# Autodesk Inventor assembly: Нога левая в сборе
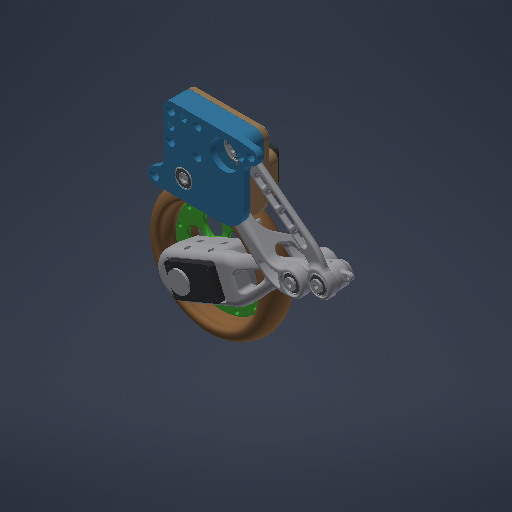
[picture p0: Inventor's stored thumbnail of the model, 512x512]
Saved by Autodesk Inventor 2025 (Build 290162010, 162A)
## iProperties
Created: 2024-06-21
Part Number: Нога левая в сборе
Document SubType Name: Assembly
Designer: Edward_Higgins
Author: Edward_Higgins
## Documents named in this file (14)
- D:\Users\Edward_Higgins\Desktop\ZAVOD\TWR2\Нога левая в сборе 2.iam
- D:\Users\Edward_Higgins\Desktop\ZAVOD\TWR2\Тяга передняя.ipt
- D:\Users\Edward_Higgins\Desktop\ZAVOD\TWR2\Стандартные детали\DYNAMIXEL XM430-W350.ipt
- D:\Users\Edward_Higgins\Desktop\ZAVOD\TWR2\Тяга задняя 2.ipt
- D:\Users\Edward_Higgins\Desktop\ZAVOD\TWR2\Голень в сборе.iam
- D:\Users\Edward_Higgins\Desktop\ZAVOD\TWR2\Стандартные детали\Подшипник.ipt
- D:\Users\Edward_Higgins\Desktop\ZAVOD\TWR2\Стопорная шайба.ipt
- D:\Users\Edward_Higgins\Desktop\ZAVOD\TWR2\Шайба.ipt
- D:\Users\Edward_Higgins\Desktop\ZAVOD\TWR2\Ось односторонняя.ipt
- D:\Users\Edward_Higgins\Desktop\ZAVOD\TWR2\Колесо 2 в сборе.iam
- D:\Users\Edward_Higgins\Desktop\ZAVOD\TWR2\Корпус ноги в сборе.iam
- D:\Users\Edward_Higgins\Desktop\ZAVOD\TWR2\Ось шарнира.ipt
- D:\Users\Edward_Higgins\Desktop\ZAVOD\TWR2\Ось двусторонняя.ipt
- D:\Users\Edward_Higgins\Desktop\ZAVOD\Робот Сколково\Нога левая в сборе\AIP\FEA\ew5x1yt6p.fres
## Components (19 placed, 12 different names)
1. Тяга передняя:1 — Совмещение:21, Совмещение:84, Совмещение:85, Совмещение:103, Совмещение:113, Совмещение:115, Совмещение:121, Совмещение:124, Совмещение:129, Совмещение:137
2. DYNAMIXEL XM430-W350:2 — Совмещение:21, Совмещение:84, Угол:1, Совмещение:104
3. Голень в сборе:1 [sub-assembly] — Совмещение:85, Совмещение:99, Совмещение:100, Совмещение:105, Совмещение:116, Совмещение:121, Совмещение:122
4. Подшипник:1 — Совмещение:110
5. Стопорная шайба:1
6. Шайба:1 — Совмещение:96, Совмещение:109
7. Ось односторонняя:1 — Совмещение:96, Совмещение:107, Совмещение:108
8. Колесо 2 в сборе:1 [sub-assembly] — Совмещение:99, Совмещение:100
9. Корпус ноги в сборе:1 [sub-assembly] — Совмещение:101, Совмещение:102, Совмещение:103, Угол:1, Совмещение:104, Совмещение:107, Совмещение:108, Совмещение:109
10. Тяга задняя 2:3 — Совмещение:105, Совмещение:110, Совмещение:119, Совмещение:120
11. Ось шарнира:1 — Совмещение:113, Совмещение:115, Совмещение:136, Совмещение:137
12. Подшипник:2 — Совмещение:116, Совмещение:117, Совмещение:118, Совмещение:119, Совмещение:120
13. Стопорная шайба:2 — Совмещение:117, Совмещение:118
14. Подшипник:3 — Совмещение:128, Совмещение:129, Совмещение:130, Совмещение:131
15. Стопорная шайба:3 — Совмещение:130, Совмещение:131
16. Подшипник:4 — Совмещение:123, Совмещение:124, Совмещение:125, Совмещение:126, Совмещение:127
17. Стопорная шайба:4 — Совмещение:126, Совмещение:127
18. Ось двусторонняя:1 — Совмещение:122, Совмещение:123, Совмещение:125, Совмещение:128
19. Подшипник:6 — Совмещение:136
## Relationships (41: Mate 40, Angle 1)
- Совмещение:21 [Mate]: Тяга передняя:1 ↔ DYNAMIXEL XM430-W350:2
- Совмещение:84 [Mate]: Тяга передняя:1 ↔ DYNAMIXEL XM430-W350:2
- Совмещение:85 [Mate]: Тяга передняя:1 ↔ Голень в сборе:1
- [Mate]: Подшипник:1 ↔ Стопорная шайба:1
- [Mate]: Подшипник:1 ↔ Стопорная шайба:1
- [Mate]: Подшипник:1 ↔ Ось односторонняя:1
- [Mate]: Подшипник:1 ↔ Ось односторонняя:1
- [Mate]: Шайба:1 ↔ Ось односторонняя:1
- Совмещение:96 [Mate]: Шайба:1 ↔ Ось односторонняя:1
- Совмещение:99 [Mate]: Голень в сборе:1 ↔ Колесо 2 в сборе:1
- Совмещение:100 [Mate]: Голень в сборе:1 ↔ Колесо 2 в сборе:1
- Совмещение:101 [Mate]: Корпус ноги в сборе:1
- Совмещение:102 [Mate]: Корпус ноги в сборе:1
- Совмещение:103 [Mate]: Тяга передняя:1 ↔ Корпус ноги в сборе:1
- Угол:1 [Angle] (0 deg): DYNAMIXEL XM430-W350:2 ↔ Корпус ноги в сборе:1
- Совмещение:104 [Mate]: DYNAMIXEL XM430-W350:2 ↔ Корпус ноги в сборе:1
- Совмещение:105 [Mate]: Голень в сборе:1 ↔ Тяга задняя 2:3
- Совмещение:107 [Mate]: Ось односторонняя:1 ↔ Корпус ноги в сборе:1
- Совмещение:108 [Mate]: Ось односторонняя:1 ↔ Корпус ноги в сборе:1
- Совмещение:109 [Mate]: Шайба:1 ↔ Корпус ноги в сборе:1
- Совмещение:110 [Mate]: Подшипник:1 ↔ Тяга задняя 2:3
- Совмещение:113 [Mate]: Тяга передняя:1 ↔ Ось шарнира:1
- Совмещение:115 [Mate]: Тяга передняя:1 ↔ Ось шарнира:1
- Совмещение:116 [Mate]: Голень в сборе:1 ↔ Подшипник:2
- Совмещение:117 [Mate]: Подшипник:2 ↔ Стопорная шайба:2
- Совмещение:118 [Mate]: Подшипник:2 ↔ Стопорная шайба:2
- Совмещение:119 [Mate]: Тяга задняя 2:3 ↔ Подшипник:2
- Совмещение:120 [Mate]: Тяга задняя 2:3 ↔ Подшипник:2
- Совмещение:121 [Mate]: Тяга передняя:1 ↔ Голень в сборе:1
- Совмещение:122 [Mate]: Голень в сборе:1 ↔ Ось двусторонняя:1
- Совмещение:123 [Mate]: Подшипник:4 ↔ Ось двусторонняя:1
- Совмещение:124 [Mate]: Тяга передняя:1 ↔ Подшипник:4
- Совмещение:125 [Mate]: Подшипник:4 ↔ Ось двусторонняя:1
- Совмещение:126 [Mate]: Подшипник:4 ↔ Стопорная шайба:4
- Совмещение:127 [Mate]: Подшипник:4 ↔ Стопорная шайба:4
- Совмещение:128 [Mate]: Подшипник:3 ↔ Ось двусторонняя:1
- Совмещение:129 [Mate]: Тяга передняя:1 ↔ Подшипник:3
- Совмещение:130 [Mate]: Подшипник:3 ↔ Стопорная шайба:3
- Совмещение:131 [Mate]: Подшипник:3 ↔ Стопорная шайба:3
- Совмещение:136 [Mate]: Ось шарнира:1 ↔ Подшипник:6
- Совмещение:137 [Mate]: Тяга передняя:1 ↔ Ось шарнира:1
## Named parameters: d26_d24 = 0 mm, d27_d25 = 0 mm
